# Autodesk Inventor assembly: Assembly1
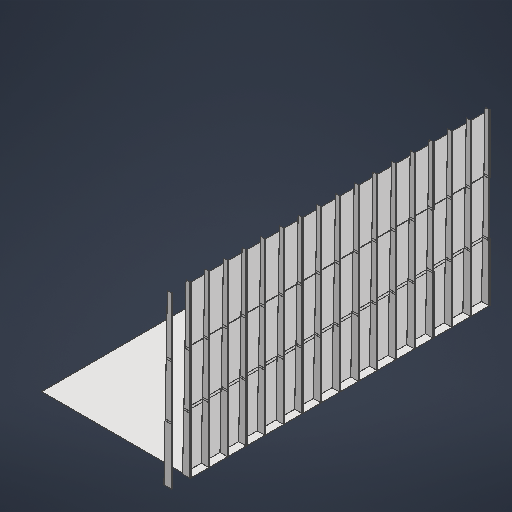
[picture p0: Inventor's stored thumbnail of the model, 512x512]
Saved by Autodesk Inventor 2026.2 (Build 302298000, 298)
## iProperties
Created: 2026-04-17
Part Number: Assembly1
Document SubType Name: Assembly
Designer: admin
Author: admin
## Documents named in this file (6)
- C:\Users\admin\Documents\Inventor\GBK-Gubkinskiy\Assembly1.iam
- C:\Users\admin\Documents\Inventor\GBK-Gubkinskiy\Part1.ipt
- C:\Users\admin\Documents\Inventor\GBK-Gubkinskiy\Part2.ipt
- C:\Users\admin\Documents\Inventor\GBK-Gubkinskiy\Part2_CPY.ipt
- C:\Users\admin\Documents\Inventor\GBK-Gubkinskiy\Part2_CPY_CPY.ipt
- C:\Users\admin\Documents\Inventor\GBK-Gubkinskiy\Part111.ipt
## Components (58 placed, 5 different names)
1. Part1:1 — Rigid:1, Flush:1, Mate:4
2. Part111:1 — Flush:1, Mate:3, Mate:4, Mate:5
3. Part111:2 — Flush:2, Mate:5, Mate:6, Flush:3
4. Part111:3 — Mate:6, Flush:3
5. Part2:1 — Rigid:1, Rigid:2, Mate:3
6. Part2_CPY:1 — Rigid:2, Rigid:3, Flush:2
7. Part2_CPY_CPY:1 — Rigid:3
8. Part2:2
9. Part2_CPY:2
10. Part2_CPY_CPY:2
11. Part2:3
12. Part2_CPY:3
13. Part2_CPY_CPY:3
14. Part2:4
15. Part2_CPY:4
16. Part2_CPY_CPY:4
17. Part2:5
18. Part2_CPY:5
19. Part2_CPY_CPY:5
20. Part2:6
21. Part2_CPY:6
22. Part2_CPY_CPY:6
23. Part2:7
24. Part2_CPY:7
25. Part2_CPY_CPY:7
26. Part2:8
27. Part2_CPY:8
28. Part2_CPY_CPY:8
29. Part2:9
30. Part2_CPY:9
31. Part2_CPY_CPY:9
32. Part2:10
33. Part2_CPY:10
34. Part2_CPY_CPY:10
35. Part2:11
36. Part2_CPY:11
37. Part2_CPY_CPY:11
38. Part2:12
39. Part2_CPY:12
40. Part2_CPY_CPY:12
41. Part2:13
42. Part2_CPY:13
43. Part2_CPY_CPY:13
44. Part2:14
45. Part2_CPY:14
46. Part2_CPY_CPY:14
47. Part2:15
48. Part2_CPY:15
49. Part2_CPY_CPY:15
50. Part2:16
51. Part2_CPY:16
52. Part2_CPY_CPY:16
53. Part2:17
54. Part2_CPY:17
55. Part2_CPY_CPY:17
56. Part2:18
57. Part2_CPY:18
58. Part2_CPY_CPY:18
## Component patterns: (18 elements, first: Part2:1 + Part2_CPY:1 + Part2_CPY_CPY:1)
## Relationships (10: Mate 4, WeldJoint 3, Flush 3)
- Rigid:1 [WeldJoint]: Part1:1 ↔ Part2:1
- Rigid:2 [WeldJoint] (-50 mm): Part2:1 ↔ Part2_CPY:1
- Rigid:3 [WeldJoint] (-50 mm): Part2_CPY:1 ↔ Part2_CPY_CPY:1
- Flush:1: Part1:1 ↔ Part111:1
- Mate:3: Part111:1 ↔ Part2:1
- Mate:4: Part1:1 ↔ Part111:1
- Flush:2: Part111:2 ↔ Part2_CPY:1
- Mate:5: Part111:1 ↔ Part111:2
- Mate:6: Part111:2 ↔ Part111:3
- Flush:3: Part111:2 ↔ Part111:3
